# Autodesk Inventor assembly: 总装配
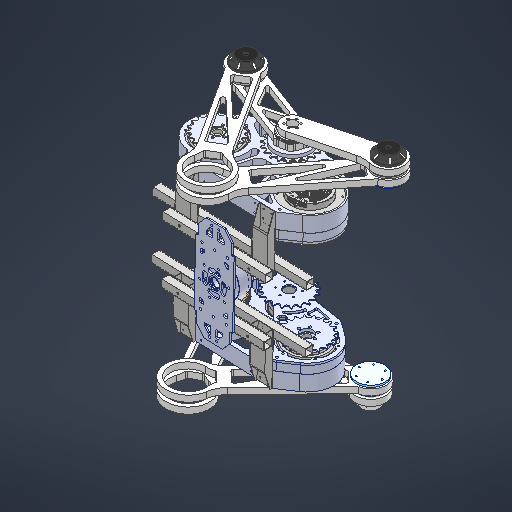
[picture p0: Inventor's stored thumbnail of the model, 512x512]
Saved by Autodesk Inventor 2025 (Build 290162000, 162)
## iProperties
Created: 2025-04-19
Part Number: 总装配
Document SubType Name: Assembly
Designer: XH
Author: XH
## Documents named in this file (10)
- C:\Users\HZD\Desktop\RCInventor\铝件版本\总装配.iam
- C:\Users\HZD\Desktop\RCInventor\铝件版本\装配体2.iam
- C:\Users\HZD\Desktop\RCInventor\铝件版本\铝方管\40x15.ipt
- C:\Users\HZD\Desktop\RCInventor\铝件版本\铝方管\15x15.ipt
- C:\Users\HZD\Desktop\RCInventor\铝件版本\GM6020 直流无刷电机_3.2.ipt
- C:\Users\HZD\Desktop\RCInventor\铝件版本\板材_云台连接板3.ipt
- C:\Users\HZD\Desktop\RCInventor\铝件版本\装配体2_MIR1.iam
- C:\Users\HZD\Desktop\RCInventor\铝件版本\铝方管\40x15_MIR.ipt
- C:\Users\HZD\Desktop\RCInventor\铝件版本\铝方管\15x15_MIR.ipt
- C:\Users\HZD\Desktop\RCInventor\铝件版本\铝方管\15x152.ipt
## Components (12 placed, 9 different names)
1. 装配体2:1 [sub-assembly] — 配合:1, 表面齐平:2, 表面齐平:3, 配合:2, 表面齐平:4, 配合:3
2. 40x15:1 — 配合:1, 表面齐平:2, 表面齐平:3, 配合:4, 表面齐平:5
3. 40x15:2 — 配合:2, 表面齐平:4, 配合:3, 配合:15, 表面齐平:17
4. 15x15:1 — 配合:4, 表面齐平:5, 表面齐平:12, 配合:16
5. GM6020 直流无刷电机_3.2:1 — 配合:5, 配合:6, 配合:7
6. 板材_云台连接板3:1 — 配合:5, 配合:6, 配合:7, 配合:17, 配合:21, 表面齐平:15, 表面齐平:16
7. 装配体2_MIR1:1 [sub-assembly] — 表面齐平:7, 表面齐平:8, 配合:10, 配合:11, 表面齐平:9, 配合:12
8. 40x15_MIR:1 — 表面齐平:7, 表面齐平:8, 配合:10, 表面齐平:10, 配合:13, 配合:19
9. 40x15_MIR:2 — 配合:11, 表面齐平:9, 配合:12, 表面齐平:17
10. 15x15_MIR:1 — 表面齐平:10, 配合:13, 配合:18, 配合:20
11. 15x152:1 — 配合:15, 表面齐平:12, 配合:16, 配合:17, 表面齐平:13, 表面齐平:14, 表面齐平:16
12. 15x152:2 — 配合:18, 配合:19, 配合:20, 表面齐平:13, 表面齐平:14, 配合:21, 表面齐平:15
## Relationships (33: Mate 18, Flush 15)
- 表面齐平:1 [Flush] (138 mm)
- 配合:1 [Mate]: 装配体2:1 ↔ 40x15:1
- 表面齐平:2 [Flush]: 装配体2:1 ↔ 40x15:1
- 表面齐平:3 [Flush]: 装配体2:1 ↔ 40x15:1
- 配合:2 [Mate]: 装配体2:1 ↔ 40x15:2
- 表面齐平:4 [Flush]: 装配体2:1 ↔ 40x15:2
- 配合:3 [Mate]: 装配体2:1 ↔ 40x15:2
- 配合:4 [Mate]: 40x15:1 ↔ 15x15:1
- 表面齐平:5 [Flush]: 40x15:1 ↔ 15x15:1
- 配合:5 [Mate]: GM6020 直流无刷电机_3.2:1 ↔ 板材_云台连接板3:1
- 配合:6 [Mate]: GM6020 直流无刷电机_3.2:1 ↔ 板材_云台连接板3:1
- 配合:7 [Mate]: GM6020 直流无刷电机_3.2:1 ↔ 板材_云台连接板3:1
- 表面齐平:7 [Flush]: 装配体2_MIR1:1 ↔ 40x15_MIR:1
- 表面齐平:8 [Flush]: 装配体2_MIR1:1 ↔ 40x15_MIR:1
- 配合:10 [Mate]: 装配体2_MIR1:1 ↔ 40x15_MIR:1
- 配合:11 [Mate]: 装配体2_MIR1:1 ↔ 40x15_MIR:2
- 表面齐平:9 [Flush]: 装配体2_MIR1:1 ↔ 40x15_MIR:2
- 配合:12 [Mate]: 装配体2_MIR1:1 ↔ 40x15_MIR:2
- 表面齐平:10 [Flush]: 40x15_MIR:1 ↔ 15x15_MIR:1
- 配合:13 [Mate]: 40x15_MIR:1 ↔ 15x15_MIR:1
- 配合:15 [Mate]: 40x15:2 ↔ 15x152:1
- 表面齐平:12 [Flush]: 15x15:1 ↔ 15x152:1
- 配合:16 [Mate]: 15x15:1 ↔ 15x152:1
- 配合:17 [Mate]: 板材_云台连接板3:1 ↔ 15x152:1
- 配合:18 [Mate]: 15x15_MIR:1 ↔ 15x152:2
- 配合:19 [Mate]: 40x15_MIR:1 ↔ 15x152:2
- 配合:20 [Mate]: 15x15_MIR:1 ↔ 15x152:2
- 表面齐平:13 [Flush]: 15x152:1 ↔ 15x152:2
- 表面齐平:14 [Flush]: 15x152:1 ↔ 15x152:2
- 配合:21 [Mate]: 板材_云台连接板3:1 ↔ 15x152:2
- 表面齐平:15 [Flush]: 板材_云台连接板3:1 ↔ 15x152:2
- 表面齐平:16 [Flush]: 板材_云台连接板3:1 ↔ 15x152:1
- 表面齐平:17 [Flush]: 40x15:2 ↔ 40x15_MIR:2
